# Autodesk Inventor assembly: 000-dribl-v1
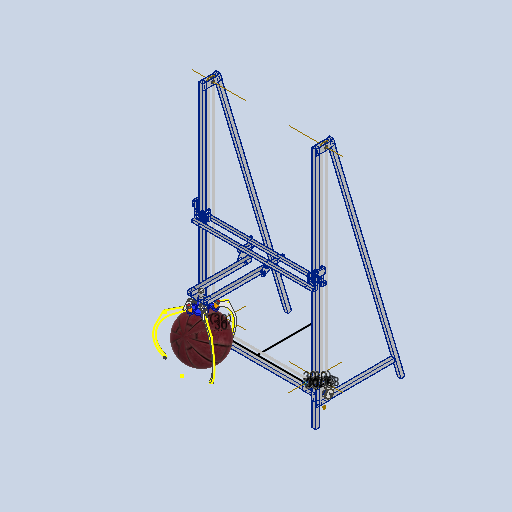
[picture p0: Inventor's stored thumbnail of the model, 512x512]
Saved by Autodesk Inventor 2025.2 (Build 292293000, 293)
## iProperties
Created: 2025-01-04
Part Number: 000-dribl-v1
Document SubType Name: Assembly
Designer: haruy
Author: haruy
## Documents named in this file (26)
- C:\Users\haruy\Documents\ロボコン\NHK2025\cad\nagahisa\dribl\000-dribl-v1.iam
- C:\Users\haruy\Documents\ロボコン\NHK2025\cad\nagahisa\dribl\dribl-v1-ASP-Base.ipt
- C:\Users\haruy\Documents\ロボコン\NHK2025\cad\nagahisa\dribl\RZvector-Srunit-v3-ASP-Base.ipt
- C:\Users\haruy\Documents\ロボコン\NHK2025\cad\nagahisa\dribl\dribl-v1-Plate-1.ipt
- C:\Users\haruy\Documents\ロボコン\NHK2025\cad\nagahisa\hand\grab\000-hand-grab-v4.iam
- C:\Users\haruy\Documents\ロボコン\NHK2025\cad\nagahisa\dribl\dribl-v1-Plate-2.ipt
- C:\Users\haruy\Documents\ロボコン\NHK2025\cad\nagahisa\dribl\dribl-v1-Plate-3.ipt
- C:\Users\haruy\Documents\ロボコン\NHK2025\cad\000_parts\モーター\robomaster\M3508.ipt
- C:\Users\haruy\Documents\ロボコン\NHK2025\cad\nagahisa\dribl\dribl-v1-Plate-4.ipt
- C:\Users\haruy\Documents\ロボコン\NHK2025\cad\nagahisa\dribl\dribl-v1-Plate-5.ipt
- C:\Users\haruy\Documents\ロボコン\NHK2025\cad\nagahisa\dribl\R2-Rzvector\TH22_bearing_12_18_19.5_sn.ipt
- C:\Users\haruy\Documents\ロボコン\NHK2025\cad\nagahisa\dribl\R2-Rzvector\MTP16XL025-A-N12.iam
- C:\Users\haruy\Documents\ロボコン\NHK2025\cad\nagahisa\dribl\dribl-v1-Shaft-1.ipt
- C:\Users\haruy\Documents\ロボコン\NHK2025\cad\nagahisa\dribl\SMB1_5-20_SMB1_5-20_On.iam
- C:\Users\haruy\Documents\ロボコン\NHK2025\cad\nagahisa\dribl\000-dribl-v1\デザイン アクセラレータ\歯付きベルト伝達1.iam
- C:\Users\haruy\Documents\ロボコン\NHK2025\cad\nagahisa\belt_liner\SCSWJ10-6.iam
- C:\Users\haruy\Documents\ロボコン\NHK2025\cad\nagahisa\dribl\000-dribl-v1\デザイン アクセラレータ\平歯車1.iam
- C:\Users\haruy\Documents\ロボコン\NHK2025\cad\nagahisa\dribl\R2-Rzvector\SCSWJ12-6.iam
- C:\Users\haruy\Documents\ロボコン\NHK2025\cad\nagahisa\dribl\000-dribl-v1\デザイン アクセラレータ\平歯車2.iam
- C:\Users\haruy\Documents\ロボコン\NHK2025\cad\nagahisa\dribl\R2-Rzvector\bear_f8_12_sa.ipt
- C:\Users\haruy\Documents\ロボコン\NHK2025\cad\nagahisa\dribl\R2-Rzvector\ATP16XL025-A-P8.iam
- C:\Users\haruy\Documents\ロボコン\NHK2025\cad\nagahisa\dribl\dribl-v1-Plate-6.ipt
- C:\Users\haruy\Documents\ロボコン\NHK2025\cad\nagahisa\dribl\R2-Rzvector\bear_10_15_sn.ipt
- C:\Users\haruy\Documents\ロボコン\NHK2025\cad\nagahisa\dribl\R2-Rzvector\ATP16XL025-A-N10.iam
- C:\Users\haruy\Documents\ロボコン\NHK2025\cad\nagahisa\dribl\000-dribl-v1\デザイン アクセラレータ\歯付きベルト伝達2.iam
- C:\Users\haruy\Documents\ロボコン\NHK2025\cad\nagahisa\dribl\000-dribl-v1\デザイン アクセラレータ\歯付きベルト伝達3.iam
## Components (49 placed, 22 different names)
1. dribl-v1-ASP-Base:1 — 正接:1, 正接:2, 正接:3, 正接:4, 正接:5, 挿入:6, 挿入:7, 挿入:8, 挿入:9, 挿入:10, 挿入:11, 挿入:12, 挿入:13, 挿入:14, 挿入:15, 挿入:17, 挿入:18, 挿入:19, 挿入:20, 挿入:21, 挿入:22, 挿入:43, 挿入:44, 挿入:45, 挿入:46, 挿入:47, 挿入:48, 挿入:49, 挿入:50
2. RZvector-Srunit-v3-ASP-Base:1 — 正接:1, 正接:2, 正接:3, 挿入:1, 挿入:2, 挿入:3, 挿入:4, 正接:4, 角度:1, 正接:5
3. dribl-v1-Plate-1:1 — 挿入:1, 挿入:2, 挿入:5
4. dribl-v1-Plate-1:2 — 挿入:3, 挿入:4
5. 000-hand-grab-v4:1 [sub-assembly] — 挿入:5, 角度:1
6. dribl-v1-Plate-2:1 — 挿入:6, 挿入:7, 挿入:27
7. dribl-v1-Plate-2:2 — 挿入:10, 挿入:11, 挿入:25
8. dribl-v1-Plate-2:3 — 挿入:12, 挿入:13, 挿入:28
9. dribl-v1-Plate-2:4 — 挿入:8, 挿入:9, 挿入:26
10. dribl-v1-Plate-3:1 — 挿入:14, 挿入:15, 挿入:16, 挿入:23
11. M3508:1 — 挿入:16, 挿入:38, メイト:1
12. dribl-v1-Plate-4:1 — 挿入:17, 挿入:18, 挿入:24, 角度:2
13. dribl-v1-Plate-5:1 — 挿入:19, 挿入:20, 挿入:29, メイト:6, 挿入:41
14. dribl-v1-Plate-5:2 — 挿入:21, 挿入:22, 挿入:30, 角度:3, 挿入:40
15. TH22_bearing_12_18_19.5_sn:1 — 挿入:23, メイト:3
16. TH22_bearing_12_18_19.5_sn:2 — 挿入:24, 挿入:31
17. TH22_bearing_12_18_19.5_sn:3 — 挿入:25, 挿入:32, 挿入:36
18. TH22_bearing_12_18_19.5_sn:4 — 挿入:26, 挿入:34
19. TH22_bearing_12_18_19.5_sn:5 — 挿入:28, 挿入:33, 挿入:37
20. TH22_bearing_12_18_19.5_sn:6 — 挿入:27, 挿入:35
21. TH22_bearing_12_18_19.5_sn:7 — 挿入:29, 挿入:39
22. TH22_bearing_12_18_19.5_sn:8 — 挿入:30
23. MTP16XL025-A-N12:1 [sub-assembly] — 挿入:31
24. MTP16XL025-A-N12:2 [sub-assembly] — 挿入:33
25. MTP16XL025-A-N12:3 [sub-assembly] — 挿入:32, フラッシュ:1
26. dribl-v1-Shaft-1:1 — 挿入:34
27. dribl-v1-Shaft-1:2 — 挿入:35
28. SMB1_5-20_SMB1_5-20_On:1 [sub-assembly] — 挿入:36, 角度:2
29. SMB1_5-20_SMB1_5-20_On:2 [sub-assembly] — 挿入:37, 角度:3
30. 歯付きベルト伝達:1 [sub-assembly]
31. SCSWJ10-6:1 [sub-assembly] — 挿入:38, メイト:2
32. 平歯車:1 [sub-assembly] — メイト:1, メイト:2, メイト:3
33. SCSWJ12-6:1 [sub-assembly] — 挿入:39, メイト:4, メイト:5
34. 平歯車:2 [sub-assembly] — メイト:4, メイト:5, メイト:6
35. bear_f8_12_sa:1 — 挿入:41
36. bear_f8_12_sa:2 — 挿入:40, 挿入:42
37. ATP16XL025-A-P8:1 [sub-assembly] — 挿入:42
38. dribl-v1-Plate-6:1 — 挿入:43, 挿入:44, 挿入:52
39. dribl-v1-Plate-6:2 — 挿入:45, 挿入:46, 挿入:51
40. dribl-v1-Plate-6:3 — 挿入:49, 挿入:50, 挿入:53
41. dribl-v1-Plate-6:4 — 挿入:47, 挿入:48, 挿入:54
42. bear_10_15_sn:1 — 挿入:52
43. bear_10_15_sn:2 — 挿入:51, 挿入:55
44. bear_10_15_sn:3 — 挿入:54
45. bear_10_15_sn:4 — 挿入:53, 挿入:56
46. ATP16XL025-A-N10:1 [sub-assembly] — 挿入:56, フラッシュ:3
47. ATP16XL025-A-N10:2 [sub-assembly] — 挿入:55, フラッシュ:2
48. 歯付きベルト伝達:2 [sub-assembly]
49. 歯付きベルト伝達:3 [sub-assembly]
## Relationships (73: Insert 56, Mate 6, Tangent 5, Angle 3, Flush 3)
- 正接:1 [Tangent]: dribl-v1-ASP-Base:1 ↔ RZvector-Srunit-v3-ASP-Base:1
- 正接:2 [Tangent]: dribl-v1-ASP-Base:1 ↔ RZvector-Srunit-v3-ASP-Base:1
- 正接:3 [Tangent]: dribl-v1-ASP-Base:1 ↔ RZvector-Srunit-v3-ASP-Base:1
- 挿入:1 [Insert]: RZvector-Srunit-v3-ASP-Base:1 ↔ dribl-v1-Plate-1:1
- 挿入:2 [Insert]: RZvector-Srunit-v3-ASP-Base:1 ↔ dribl-v1-Plate-1:1
- 挿入:3 [Insert]: RZvector-Srunit-v3-ASP-Base:1 ↔ dribl-v1-Plate-1:2
- 挿入:4 [Insert]: RZvector-Srunit-v3-ASP-Base:1 ↔ dribl-v1-Plate-1:2
- 挿入:5 [Insert] (10 mm): dribl-v1-Plate-1:1 ↔ 000-hand-grab-v4:1
- 正接:4 [Tangent]: dribl-v1-ASP-Base:1 ↔ RZvector-Srunit-v3-ASP-Base:1
- 角度:1 [Angle] (0 deg): RZvector-Srunit-v3-ASP-Base:1 ↔ 000-hand-grab-v4:1
- 正接:5 [Tangent]: dribl-v1-ASP-Base:1 ↔ RZvector-Srunit-v3-ASP-Base:1
- 挿入:6 [Insert]: dribl-v1-ASP-Base:1 ↔ dribl-v1-Plate-2:1
- 挿入:7 [Insert]: dribl-v1-ASP-Base:1 ↔ dribl-v1-Plate-2:1
- 挿入:8 [Insert]: dribl-v1-ASP-Base:1 ↔ dribl-v1-Plate-2:4
- 挿入:9 [Insert]: dribl-v1-ASP-Base:1 ↔ dribl-v1-Plate-2:4
- 挿入:10 [Insert]: dribl-v1-ASP-Base:1 ↔ dribl-v1-Plate-2:2
- 挿入:11 [Insert]: dribl-v1-ASP-Base:1 ↔ dribl-v1-Plate-2:2
- 挿入:12 [Insert]: dribl-v1-ASP-Base:1 ↔ dribl-v1-Plate-2:3
- 挿入:13 [Insert]: dribl-v1-ASP-Base:1 ↔ dribl-v1-Plate-2:3
- 挿入:14 [Insert]: dribl-v1-ASP-Base:1 ↔ dribl-v1-Plate-3:1
- 挿入:15 [Insert]: dribl-v1-ASP-Base:1 ↔ dribl-v1-Plate-3:1
- 挿入:16 [Insert]: dribl-v1-Plate-3:1 ↔ M3508:1
- 挿入:17 [Insert]: dribl-v1-ASP-Base:1 ↔ dribl-v1-Plate-4:1
- 挿入:18 [Insert]: dribl-v1-ASP-Base:1 ↔ dribl-v1-Plate-4:1
- 挿入:19 [Insert]: dribl-v1-ASP-Base:1 ↔ dribl-v1-Plate-5:1
- 挿入:20 [Insert]: dribl-v1-ASP-Base:1 ↔ dribl-v1-Plate-5:1
- 挿入:21 [Insert]: dribl-v1-ASP-Base:1 ↔ dribl-v1-Plate-5:2
- 挿入:22 [Insert]: dribl-v1-ASP-Base:1 ↔ dribl-v1-Plate-5:2
- 挿入:23 [Insert]: dribl-v1-Plate-3:1 ↔ TH22_bearing_12_18_19.5_sn:1
- 挿入:24 [Insert]: dribl-v1-Plate-4:1 ↔ TH22_bearing_12_18_19.5_sn:2
- 挿入:25 [Insert]: dribl-v1-Plate-2:2 ↔ TH22_bearing_12_18_19.5_sn:3
- 挿入:26 [Insert]: dribl-v1-Plate-2:4 ↔ TH22_bearing_12_18_19.5_sn:4
- 挿入:27 [Insert]: dribl-v1-Plate-2:1 ↔ TH22_bearing_12_18_19.5_sn:6
- 挿入:28 [Insert]: dribl-v1-Plate-2:3 ↔ TH22_bearing_12_18_19.5_sn:5
- 挿入:29 [Insert]: dribl-v1-Plate-5:1 ↔ TH22_bearing_12_18_19.5_sn:7
- 挿入:30 [Insert]: dribl-v1-Plate-5:2 ↔ TH22_bearing_12_18_19.5_sn:8
- 挿入:31 [Insert] (2.75 mm): TH22_bearing_12_18_19.5_sn:2 ↔ MTP16XL025-A-N12:1
- 挿入:32 [Insert] (2.75 mm): TH22_bearing_12_18_19.5_sn:3 ↔ MTP16XL025-A-N12:3
- 挿入:33 [Insert] (2.75 mm): TH22_bearing_12_18_19.5_sn:5 ↔ MTP16XL025-A-N12:2
- 挿入:34 [Insert]: TH22_bearing_12_18_19.5_sn:4 ↔ dribl-v1-Shaft-1:1
- 挿入:35 [Insert]: TH22_bearing_12_18_19.5_sn:6 ↔ dribl-v1-Shaft-1:2
- 挿入:36 [Insert] (2.18 mm): TH22_bearing_12_18_19.5_sn:3 ↔ SMB1_5-20_SMB1_5-20_On:1
- 角度:2 [Angle] (0 deg): dribl-v1-Plate-4:1 ↔ SMB1_5-20_SMB1_5-20_On:1
- 挿入:37 [Insert] (2.18 mm): TH22_bearing_12_18_19.5_sn:5 ↔ SMB1_5-20_SMB1_5-20_On:2
- 角度:3 [Angle] (0 deg): dribl-v1-Plate-5:2 ↔ SMB1_5-20_SMB1_5-20_On:2
- フラッシュ:1 [Flush] (-6.25 mm): MTP16XL025-A-N12:3
- 挿入:38 [Insert] (5 mm): M3508:1 ↔ SCSWJ10-6:1
- メイト:1 [Mate]: M3508:1 ↔ 平歯車:1
- メイト:2 [Mate]: SCSWJ10-6:1 ↔ 平歯車:1
- メイト:3 [Mate]: TH22_bearing_12_18_19.5_sn:1 ↔ 平歯車:1
- 挿入:39 [Insert] (5 mm): TH22_bearing_12_18_19.5_sn:7 ↔ SCSWJ12-6:1
- メイト:4 [Mate]: SCSWJ12-6:1 ↔ 平歯車:2
- メイト:5 [Mate]: SCSWJ12-6:1 ↔ 平歯車:2
- メイト:6 [Mate]: dribl-v1-Plate-5:1 ↔ 平歯車:2
- 挿入:40 [Insert]: dribl-v1-Plate-5:2 ↔ bear_f8_12_sa:2
- 挿入:41 [Insert]: dribl-v1-Plate-5:1 ↔ bear_f8_12_sa:1
- 挿入:42 [Insert] (2.95 mm): bear_f8_12_sa:2 ↔ ATP16XL025-A-P8:1
- 挿入:43 [Insert]: dribl-v1-ASP-Base:1 ↔ dribl-v1-Plate-6:1
- 挿入:44 [Insert]: dribl-v1-ASP-Base:1 ↔ dribl-v1-Plate-6:1
- 挿入:45 [Insert]: dribl-v1-ASP-Base:1 ↔ dribl-v1-Plate-6:2
- 挿入:46 [Insert]: dribl-v1-ASP-Base:1 ↔ dribl-v1-Plate-6:2
- 挿入:47 [Insert]: dribl-v1-ASP-Base:1 ↔ dribl-v1-Plate-6:4
- 挿入:48 [Insert]: dribl-v1-ASP-Base:1 ↔ dribl-v1-Plate-6:4
- 挿入:49 [Insert]: dribl-v1-ASP-Base:1 ↔ dribl-v1-Plate-6:3
- 挿入:50 [Insert]: dribl-v1-ASP-Base:1 ↔ dribl-v1-Plate-6:3
- 挿入:51 [Insert]: dribl-v1-Plate-6:2 ↔ bear_10_15_sn:2
- 挿入:52 [Insert]: dribl-v1-Plate-6:1 ↔ bear_10_15_sn:1
- 挿入:53 [Insert]: dribl-v1-Plate-6:3 ↔ bear_10_15_sn:4
- 挿入:54 [Insert]: dribl-v1-Plate-6:4 ↔ bear_10_15_sn:3
- 挿入:55 [Insert] (2.75 mm): bear_10_15_sn:2 ↔ ATP16XL025-A-N10:2
- 挿入:56 [Insert] (2.75 mm): bear_10_15_sn:4 ↔ ATP16XL025-A-N10:1
- フラッシュ:2 [Flush] (-6.25 mm): ATP16XL025-A-N10:2
- フラッシュ:3 [Flush] (-6.25 mm): ATP16XL025-A-N10:1
